# Autodesk Inventor assembly: Motion-Bracket-With-End-Cap-Bearing
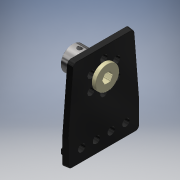
[picture p0: Inventor's stored thumbnail of the model, 180x180]
Saved by Autodesk Inventor 2017.3 (Build 213256000, 256)
## iProperties
Created: 2018-01-05
Part Number: Motion-Bracket-With-End-Cap-Bearing
Document SubType Name: Assembly
Designer: pranav
Author: pranav
## iProperties of the stored document REV-41-1327.ipt
Created: 2017-04-10
Part Number: REV-41-1327
Material: Generic
Document SubType Name: Modeling
Designer: pranav
Density: 1 g/cm^3
Appearance: Default
Sending System: Autodesk Translation Framework v5.2.0.2920
Preprocessor: ST-DEVELOPER v16.5
Title: E:/Dropbox/REV Robotics/STEP Files/REV-41-1327.step
## iProperties of the stored document REV-41-1329.ipt
Created: 2016-09-04
Part Number: REV-41-1329
Material: Generic
Description: STEP AP203
Document SubType Name: Modeling
Designer: pranav
Density: 1 g/cm^3
Appearance: Default
Sending System: SolidWorks 2015
Preprocessor: SwSTEP 2.0
Title: REV-41-1329_Default.step
Revision Number: ANY
## iProperties of the stored document REV-41-1303.ipt
Created: 2016-09-04
Part Number: REV-41-1303
Material: Generic
Description: STEP AP203
Document SubType Name: Modeling
Designer: pranav
Density: 1 g/cm^3
Appearance: Default
Mass: 4.93797 g
Surface Area: 42.214 cm^2
Volume: 4.93797 cm^3
Sending System: SolidWorks 2015
Preprocessor: SwSTEP 2.0
Title: REV-41-1303_Default.step
Revision Number: ANY
## Documents named in this file (7)
- **C:\Users\pranav\Documents\Inventor\REV-Robot-CAD\Motion-Bracket-With-End-Cap-Bearing.iam*LocalDocs*xNnihhntbS3sxu3w4Hicnix2qMd*REV-41-1327.ipt
- **C:\Users\pranav\Documents\Inventor\REV-Robot-CAD\Motion-Bracket-With-End-Cap-Bearing.iam*LocalDocs*x3zimddzbQydnevs5UxslzalzXd*REV-41-1329.ipt
- **C:\Users\pranav\Documents\Inventor\REV-Robot-CAD\Motion-Bracket-With-End-Cap-Bearing.iam*LocalDocs*xXru5gdl4Fc1ged4c4lren41uSd*REV-41-1303.ipt
- C:\Users\pranav\Documents\Inventor\REV-Robot-CAD\Motion-Bracket-With-End-Cap-Bearing.iam
- C:\Users\pranav\Documents\Inventor\REV-Robot-CAD\REV Robotics\REV Robotics CAD\REV-41-1303.step
- C:\Users\pranav\Documents\Inventor\REV-Robot-CAD\REV Robotics\REV Robotics CAD\REV-41-1329.step
- C:\Users\pranav\Documents\Inventor\REV-Robot-CAD\REV Robotics\REV Robotics CAD\REV-41-1327.step
## Components (3 placed, 3 different names)
1. REV-41-1303:1 — Mate:1, Rotational:1
2. REV-41-1329:1 — Mate:1, Rotational:1, Mate:3
3. REV-41-1327:1 — Mate:3
## Relationships (3: Mate 2, RevoluteJoint 1)
- Mate:1: REV-41-1303:1 ↔ REV-41-1329:1
- Rotational:1 [RevoluteJoint]: REV-41-1303:1 ↔ REV-41-1329:1
- Mate:3: REV-41-1329:1 ↔ REV-41-1327:1
